# Autodesk Inventor assembly: Assembly
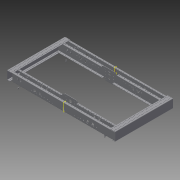
[picture p0: Inventor's stored thumbnail of the model, 180x180]
Saved by Autodesk Inventor 2015 (Build 190159000, 159)
## iProperties
Created: 2015-01-10
Part Number: Assembly
Document SubType Name: Assembly
Designer: whitaus15
Title: AM14U2 Long.STEP
Description: STEP AP203
Creation Date: 2014-12-11
Sending System: SolidWorks 2014
Preprocessor: SwSTEP 2.0
Author: whitaus15
## Documents named in this file (2)
- \\lhssvr02\Homedirs\Robotics Club\CAD Model 2015\KOP Drive Base.iam
- \\lhssvr02\Homedirs\Robotics Club\CAD Model 2015\Imported Components\AM14U2 Long\AM14U2 Half Long.iam
## Components (2 placed, 2 different names)
1. AM14U2 Half Long_1 [sub-assembly] — Flush:1
2. AM14U2 Half Long_2 [sub-assembly] — Flush:1
## Relationships (1: Flush 1)
- Flush:1: AM14U2 Half Long_1 ↔ AM14U2 Half Long_2
